# Autodesk Inventor assembly: V1Flywheel
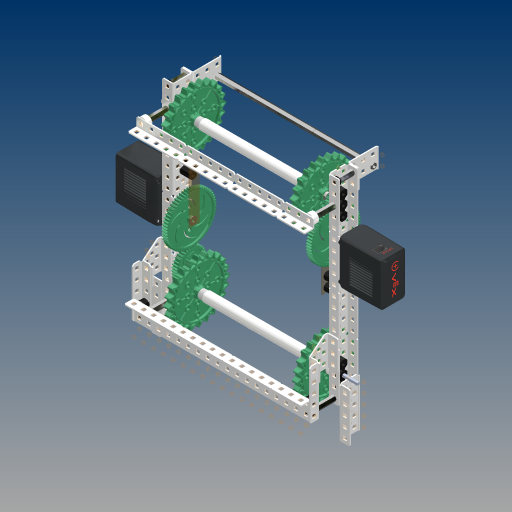
[picture p0: Inventor's stored thumbnail of the model, 512x512]
Saved by Autodesk Inventor 2023 (Build 270158000, 158)
## iProperties
Created: 2023-07-16
Part Number: V1Flywheel
Document SubType Name: Assembly
Designer: eddie
Author: eddie
## Documents named in this file (35)
- C:\Users\eddie\Documents\81208X-Over-Under-CAD\V1\V1Flywheel.iam
- C:\Users\eddie\Documents\81208X-Over-Under-CAD\VEX-CAD-Inventor-1.4.0\Structure\C Channel\Aluminum 1x2x1\Alu C 1x2x1x20.ipt
- C:\Users\eddie\Documents\81208X-Over-Under-CAD\VEX-CAD-Inventor-1.4.0\Motion\Shaft LS\Bearing Flat.ipt
- C:\Users\eddie\Documents\81208X-Over-Under-CAD\VEX-CAD-Inventor-1.4.0\Electronics\V5 Motor.ipt
- C:\Users\eddie\Documents\81208X-Over-Under-CAD\VEX-CAD-Inventor-1.4.0\Structure\Standoff\Standoff 1.00.ipt
- C:\Users\eddie\Documents\81208X-Over-Under-CAD\VEX-CAD-Inventor-1.4.0\Structure\Standoff.ipt
- C:\Users\eddie\Documents\81208X-Over-Under-CAD\VEX-CAD-Inventor-1.4.0\Motion\Spacers\Spacer Nylon .500 OD\NSpacer White .500 OD x .250.ipt
- C:\Users\eddie\Documents\81208X-Over-Under-CAD\VEX-CAD-Inventor-1.4.0\Motion\Spacers\Spacer Nylon .500 OD.ipt
- C:\Users\eddie\Documents\81208X-Over-Under-CAD\VEX-CAD-Inventor-1.4.0\Structure\Angle\Aluminum\1x1\Alu Angle 1x1x18.ipt
- C:\Users\eddie\Documents\81208X-Over-Under-CAD\VEX-CAD-Inventor-1.4.0\Motion\Shaft LS\Shaft LS\Shaft LS 9.0.ipt
- C:\Users\eddie\Documents\81208X-Over-Under-CAD\VEX-CAD-Inventor-1.4.0\Motion\Shaft LS\Shaft LS.ipt
- C:\Users\eddie\Documents\81208X-Over-Under-CAD\Custom-parts\Shaft Collar.ipt
- C:\Users\eddie\Documents\81208X-Over-Under-CAD\VEX-CAD-Inventor-1.4.0\Motion\Sprockets\9P Sprocket\9P 24T Sprocket, Square.iam
- C:\Users\eddie\Documents\81208X-Over-Under-CAD\VEX-CAD-Inventor-1.4.0\Motion\Sprockets\9P Sprocket.iam
- C:\Users\eddie\Documents\81208X-Over-Under-CAD\VEX-CAD-Inventor-1.4.0\Motion\Spacers\Spacer Nylon .500 OD\NSpacer White .500 OD x .375.ipt
- C:\Users\eddie\Documents\81208X-Over-Under-CAD\VEX-CAD-Inventor-1.4.0\Motion\Spacers\Washer Steel\SWasher .375 OD x .031250.ipt
- C:\Users\eddie\Documents\81208X-Over-Under-CAD\VEX-CAD-Inventor-1.4.0\Motion\Spacers\Washer Steel.ipt
- C:\Users\eddie\Documents\81208X-Over-Under-CAD\VEX-CAD-Inventor-1.4.0\Motion\Gears\LS 12T Gear.ipt
- C:\Users\eddie\Documents\81208X-Over-Under-CAD\VEX-CAD-Inventor-1.4.0\Motion\Gears\LS 60T Gear.ipt
- C:\Users\eddie\Documents\81208X-Over-Under-CAD\VEX-CAD-Inventor-1.4.0\Motion\Spacers\Spacer Nylon .375 OD\NSpacer .375 OD x .125.ipt
- C:\Users\eddie\Documents\81208X-Over-Under-CAD\VEX-CAD-Inventor-1.4.0\Motion\Spacers\Spacer Nylon .375 OD.ipt
- C:\Users\eddie\Documents\81208X-Over-Under-CAD\VEX-CAD-Inventor-1.4.0\Motion\Gears\LS 36T Gear.ipt
- C:\Users\eddie\Documents\81208X-Over-Under-CAD\VEX-CAD-Inventor-1.4.0\Motion\Gears\LS 12T Gear Steel.ipt
- C:\Users\eddie\Documents\81208X-Over-Under-CAD\VEX-CAD-Inventor-1.4.0\Structure\Angle\Aluminum\1x1\Alu Angle 1x1x5.ipt
- C:\Users\eddie\Documents\81208X-Over-Under-CAD\VEX-CAD-Inventor-1.4.0\Motion\Spacers\Spacer Nylon .375 OD\NSpacer .375 OD x .250.ipt
- C:\Users\eddie\Documents\81208X-Over-Under-CAD\Custom-parts\3x3x18 channel minus halfcut.ipt
- C:\Users\eddie\Documents\81208X-Over-Under-CAD\Custom-parts\3x2 channel triangular slice.ipt
- C:\Users\eddie\Documents\81208X-Over-Under-CAD\Custom-parts\2x3 channel without 1 side.ipt
- C:\Users\eddie\Documents\81208X-Over-Under-CAD\VEX-CAD-Inventor-1.4.0\Structure\Standoff\Standoff .75.ipt
- C:\Users\eddie\Documents\81208X-Over-Under-CAD\VEX-CAD-Inventor-1.4.0\Structure\Standoff\Standoff 5.00.ipt
- C:\Users\eddie\Documents\81208X-Over-Under-CAD\VEX-CAD-Inventor-1.4.0\Structure\Standoff\Standoff 3.00.ipt
- C:\Users\eddie\Documents\81208X-Over-Under-CAD\Custom-parts\2x5 channel without 1 side.ipt
- C:\Users\eddie\Documents\81208X-Over-Under-CAD\VEX-CAD-Inventor-1.4.0\Structure\Hardware\Nut Nylock.ipt
- C:\Users\eddie\Documents\81208X-Over-Under-CAD\Custom-parts\6holepolycarb.ipt
- C:\Users\eddie\Documents\81208X-Over-Under-CAD\VEX-CAD-Inventor-1.4.0\Motion\Spacers\Spacer Nylon .375 OD\NSpacer .375 OD x .375.ipt
## Components (119 placed, 28 different names)
1. Alu C 1x2x1x20:1 — Insert:1, Insert:2, Insert:3, Insert:36, Insert:71, Insert:72, Insert:91, Insert:92, Insert:96, Insert:119, Insert:120
2. Bearing Flat:1 — Insert:1, Insert:10
3. V5 Motor:1 — Insert:2
4. Standoff 1.00:1 — Insert:3, Insert:4
5. NSpacer White .500 OD x .250:1 — Insert:4, Insert:5
6. Alu Angle 1x1x18:1 — Insert:5, Insert:6
7. NSpacer White .500 OD x .250:2 — Insert:6, Insert:7
8. Standoff 1.00:2 — Insert:7, Insert:8
9. Alu C 1x2x1x20:2 — Insert:8, Insert:9, Insert:11, Insert:39, Insert:40, Insert:41, Insert:42, Insert:44, Insert:47, Insert:80, Insert:90, Insert:93, Insert:98, Insert:114, Mate:1
10. Bearing Flat:2 — Insert:9
11. Shaft LS 9.0:1 — Insert:10
12. NSpacer White .500 OD x .250:3 — Insert:11, Insert:12
13. Shaft Collar:1 — Insert:13, Insert:14
14. 9P 24T Sprocket, Square:1 [sub-assembly] — Insert:12, Insert:13
15. NSpacer White .500 OD x .250:4 — Insert:14, Insert:15
16. NSpacer White .500 OD x .375:5 — Insert:15, Insert:16
17. NSpacer White .500 OD x .375:6 — Insert:18, Insert:19
18. NSpacer White .500 OD x .375:7 — Insert:21, Insert:22
19. NSpacer White .500 OD x .375:8 — Insert:19, Insert:20
20. NSpacer White .500 OD x .375:9 — Insert:17, Insert:18
21. NSpacer White .500 OD x .375:10 — Insert:16, Insert:17
22. NSpacer White .500 OD x .375:11 — Insert:24, Insert:25
23. NSpacer White .500 OD x .375:12 — Insert:22, Insert:23
24. NSpacer White .500 OD x .375:13 — Insert:25, Insert:26
25. NSpacer White .500 OD x .375:14 — Insert:23, Insert:24
26. NSpacer White .500 OD x .375:15 — Insert:26, Insert:27
27. NSpacer White .500 OD x .375:16 — Insert:27, Insert:28
28. NSpacer White .500 OD x .375:17 — Insert:20, Insert:21
29. NSpacer White .500 OD x .375:18 — Insert:28, Insert:29
30. Shaft Collar:2 — Insert:29, Insert:30
31. 9P 24T Sprocket, Square:2 [sub-assembly] — Insert:30, Insert:31
32. SWasher .375 OD x .031250:1 — Insert:31, Insert:32
33. SWasher .375 OD x .031250:2 — Insert:32, Insert:33
34. SWasher .375 OD x .031250:3 — Insert:34, Insert:35
35. SWasher .375 OD x .031250:4 — Insert:33, Insert:34
36. LS 12T Gear:1 — Insert:35
37. SWasher .375 OD x .031250:5 — Insert:36, Insert:37
38. LS 60T Gear:1 — Insert:37, Insert:123
39. Bearing Flat:3 — Insert:39, Insert:46, Insert:109
40. Bearing Flat:4 — Insert:40
41. V5 Motor:2 — Insert:41
42. NSpacer .375 OD x .125:1 — Insert:42, Insert:43
43. LS 60T Gear:2 — Insert:43, Insert:112
44. LS 36T Gear:1 — Insert:45
45. NSpacer .375 OD x .125:2 — Insert:44, Insert:45
46. Shaft LS 9.0:2 — Insert:46
47. LS 12T Gear Steel:1 — Insert:47, Insert:48
48. SWasher .375 OD x .031250:6 — Insert:48, Insert:49
49. SWasher .375 OD x .031250:7 — Insert:49, Insert:50
50. 9P 24T Sprocket, Square:3 [sub-assembly] — Insert:50, Insert:51
51. Shaft Collar:3 — Insert:51, Insert:52
52. NSpacer White .500 OD x .375:19 — Insert:52, Insert:53
53. NSpacer White .500 OD x .375:20 — Insert:53, Insert:54
54. NSpacer White .500 OD x .375:21 — Insert:54, Insert:55
55. NSpacer White .500 OD x .375:22 — Insert:55, Insert:56
56. NSpacer White .500 OD x .375:23 — Insert:57, Insert:58
57. NSpacer White .500 OD x .375:24 — Insert:56, Insert:57
58. NSpacer White .500 OD x .250:25 — Insert:58, Insert:59
59. NSpacer White .500 OD x .375:26 — Insert:59, Insert:60
60. NSpacer White .500 OD x .375:27 — Insert:60, Insert:61
61. NSpacer White .500 OD x .375:28 — Insert:61, Insert:62
62. NSpacer White .500 OD x .375:29 — Insert:62, Insert:63
63. NSpacer White .500 OD x .375:30 — Insert:63, Insert:64
64. NSpacer White .500 OD x .375:31 — Insert:64, Insert:65
65. NSpacer White .500 OD x .375:32 — Insert:66, Insert:67
66. NSpacer White .500 OD x .375:33 — Insert:65, Insert:66
67. Shaft Collar:4 — Insert:67, Insert:68
68. 9P 24T Sprocket, Square:4 [sub-assembly] — Insert:68, Insert:69
69. NSpacer White .500 OD x .250:34 — Insert:69
70. Bearing Flat:5 — Insert:71, Insert:106
71. Standoff 1.00:3 — Insert:72, Insert:73
72. Alu Angle 1x1x5:1 — Insert:73, Insert:74, Insert:75
73. NSpacer .375 OD x .250:3 — Insert:76, Insert:78
74. NSpacer .375 OD x .250:4 — Insert:77, Insert:79
75. SWasher .375 OD x .031250:8 — Insert:79
76. SWasher .375 OD x .031250:9 — Insert:75, Insert:77
77. SWasher .375 OD x .031250:10 — Insert:74, Insert:76
78. SWasher .375 OD x .031250:11 — Insert:78
79. Standoff 1.00:4 — Insert:80, Insert:82
80. Alu Angle 1x1x5:2 — Insert:82, Insert:83, Insert:84
81. SWasher .375 OD x .031250:12 — Insert:84, Insert:86
82. SWasher .375 OD x .031250:13 — Insert:83, Insert:85
83. SWasher .375 OD x .031250:14 — Insert:87
84. SWasher .375 OD x .031250:15 — Insert:88, Insert:89
85. NSpacer .375 OD x .250:5 — Insert:86, Insert:88
86. NSpacer .375 OD x .250:6 — Insert:85, Insert:87
87. 3x3x18 channel minus halfcut:1 — Insert:89
88. 3x2 channel triangular slice:1 — Insert:90
89. 3x2 channel triangular slice:2 — Insert:91
90. 2x3 channel without 1 side:1 — Insert:92
91. 2x3 channel without 1 side:2 — Insert:93, Insert:100
92. NSpacer .375 OD x .125:8 — Insert:96, Insert:97
93. Standoff .75:6 — Insert:97
94. NSpacer .375 OD x .125:9 — Insert:98, Insert:99
95. Standoff .75:7 — Insert:99
96. Standoff 5.00:8 — Insert:100, Insert:101
97. Standoff 3.00:9 — Insert:101
98. 2x5 channel without 1 side:1 — Insert:108
99. Nut Nylock:1 — Insert:106, Insert:107
100. SWasher .375 OD x .031250:18 — Insert:107, Insert:108
101. Nut Nylock:2 — Insert:109, Insert:110
102. SWasher .375 OD x .031250:19 — Insert:110, Insert:111
103. 2x5 channel without 1 side:2 — Insert:111
104. SWasher .375 OD x .031250:20 — Insert:112, Insert:113
105. 6holepolycarb:1 — Insert:113
106. SWasher .375 OD x .031250:22 — Insert:114, Insert:116
107. SWasher .375 OD x .031250:24 — Mate:1, Insert:115
108. NSpacer .375 OD x .375:10 — Insert:115, Insert:118
109. NSpacer .375 OD x .375:11 — Insert:116, Insert:117
110. NSpacer .375 OD x .125:12 — Insert:118
111. NSpacer .375 OD x .125:13 — Insert:117
112. SWasher .375 OD x .031250:25 — Insert:120, Insert:122
113. SWasher .375 OD x .031250:26 — Insert:119, Insert:121
114. NSpacer .375 OD x .375:14 — Insert:121, Insert:125
115. NSpacer .375 OD x .375:15 — Insert:122, Insert:126
116. 6holepolycarb:2 — Insert:124
117. NSpacer .375 OD x .125:16 — Insert:123, Insert:124
118. NSpacer .375 OD x .125:17 — Insert:125
119. NSpacer .375 OD x .125:18 — Insert:126
## Relationships (118: Insert 117, Mate 1)
- Insert:1: Alu C 1x2x1x20:1 ↔ Bearing Flat:1
- Insert:2: Alu C 1x2x1x20:1 ↔ V5 Motor:1
- Insert:3: Alu C 1x2x1x20:1 ↔ Standoff 1.00:1
- Insert:4: Standoff 1.00:1 ↔ NSpacer White .500 OD x .250:1
- Insert:5: NSpacer White .500 OD x .250:1 ↔ Alu Angle 1x1x18:1
- Insert:6: Alu Angle 1x1x18:1 ↔ NSpacer White .500 OD x .250:2
- Insert:7: NSpacer White .500 OD x .250:2 ↔ Standoff 1.00:2
- Insert:8: Standoff 1.00:2 ↔ Alu C 1x2x1x20:2
- Insert:9: Alu C 1x2x1x20:2 ↔ Bearing Flat:2
- Insert:10: Bearing Flat:1 ↔ Shaft LS 9.0:1
- Insert:11: Alu C 1x2x1x20:2 ↔ NSpacer White .500 OD x .250:3
- Insert:12: NSpacer White .500 OD x .250:3 ↔ 9P 24T Sprocket, Square:1
- Insert:13: Shaft Collar:1 ↔ 9P 24T Sprocket, Square:1
- Insert:14: Shaft Collar:1 ↔ NSpacer White .500 OD x .250:4
- Insert:15: NSpacer White .500 OD x .250:4 ↔ NSpacer White .500 OD x .375:5
- Insert:16: NSpacer White .500 OD x .375:5 ↔ NSpacer White .500 OD x .375:10
- Insert:17: NSpacer White .500 OD x .375:9 ↔ NSpacer White .500 OD x .375:10
- Insert:18: NSpacer White .500 OD x .375:6 ↔ NSpacer White .500 OD x .375:9
- Insert:19: NSpacer White .500 OD x .375:6 ↔ NSpacer White .500 OD x .375:8
- Insert:20: NSpacer White .500 OD x .375:8 ↔ NSpacer White .500 OD x .375:17
- Insert:21: NSpacer White .500 OD x .375:7 ↔ NSpacer White .500 OD x .375:17
- Insert:22: NSpacer White .500 OD x .375:7 ↔ NSpacer White .500 OD x .375:12
- Insert:23: NSpacer White .500 OD x .375:12 ↔ NSpacer White .500 OD x .375:14
- Insert:24: NSpacer White .500 OD x .375:11 ↔ NSpacer White .500 OD x .375:14
- Insert:25: NSpacer White .500 OD x .375:11 ↔ NSpacer White .500 OD x .375:13
- Insert:26: NSpacer White .500 OD x .375:13 ↔ NSpacer White .500 OD x .375:15
- Insert:27: NSpacer White .500 OD x .375:15 ↔ NSpacer White .500 OD x .375:16
- Insert:28: NSpacer White .500 OD x .375:16 ↔ NSpacer White .500 OD x .375:18
- Insert:29: NSpacer White .500 OD x .375:18 ↔ Shaft Collar:2
- Insert:30: Shaft Collar:2 ↔ 9P 24T Sprocket, Square:2
- Insert:31: 9P 24T Sprocket, Square:2 ↔ SWasher .375 OD x .031250:1
- Insert:32: SWasher .375 OD x .031250:1 ↔ SWasher .375 OD x .031250:2
- Insert:33: SWasher .375 OD x .031250:2 ↔ SWasher .375 OD x .031250:4
- Insert:34: SWasher .375 OD x .031250:3 ↔ SWasher .375 OD x .031250:4
- Insert:35: SWasher .375 OD x .031250:3 ↔ LS 12T Gear:1
- Insert:36: Alu C 1x2x1x20:1 ↔ SWasher .375 OD x .031250:5
- Insert:37: SWasher .375 OD x .031250:5 ↔ LS 60T Gear:1
- Insert:39: Alu C 1x2x1x20:2 ↔ Bearing Flat:3
- Insert:40: Alu C 1x2x1x20:2 ↔ Bearing Flat:4
- Insert:41: Alu C 1x2x1x20:2 ↔ V5 Motor:2
- Insert:42: Alu C 1x2x1x20:2 ↔ NSpacer .375 OD x .125:1
- Insert:43: NSpacer .375 OD x .125:1 ↔ LS 60T Gear:2
- Insert:44: Alu C 1x2x1x20:2 ↔ NSpacer .375 OD x .125:2
- Insert:45: LS 36T Gear:1 ↔ NSpacer .375 OD x .125:2
- Insert:46: Bearing Flat:3 ↔ Shaft LS 9.0:2
- Insert:47: Alu C 1x2x1x20:2 ↔ LS 12T Gear Steel:1
- Insert:48: LS 12T Gear Steel:1 ↔ SWasher .375 OD x .031250:6
- Insert:49: SWasher .375 OD x .031250:6 ↔ SWasher .375 OD x .031250:7
- Insert:50: SWasher .375 OD x .031250:7 ↔ 9P 24T Sprocket, Square:3
- Insert:51: 9P 24T Sprocket, Square:3 ↔ Shaft Collar:3
- Insert:52: Shaft Collar:3 ↔ NSpacer White .500 OD x .375:19
- Insert:53: NSpacer White .500 OD x .375:19 ↔ NSpacer White .500 OD x .375:20
- Insert:54: NSpacer White .500 OD x .375:20 ↔ NSpacer White .500 OD x .375:21
- Insert:55: NSpacer White .500 OD x .375:21 ↔ NSpacer White .500 OD x .375:22
- Insert:56: NSpacer White .500 OD x .375:22 ↔ NSpacer White .500 OD x .375:24
- Insert:57: NSpacer White .500 OD x .375:23 ↔ NSpacer White .500 OD x .375:24
- Insert:58: NSpacer White .500 OD x .375:23 ↔ NSpacer White .500 OD x .250:25
- Insert:59: NSpacer White .500 OD x .250:25 ↔ NSpacer White .500 OD x .375:26
- Insert:60: NSpacer White .500 OD x .375:26 ↔ NSpacer White .500 OD x .375:27
- Insert:61: NSpacer White .500 OD x .375:27 ↔ NSpacer White .500 OD x .375:28
- Insert:62: NSpacer White .500 OD x .375:28 ↔ NSpacer White .500 OD x .375:29
- Insert:63: NSpacer White .500 OD x .375:29 ↔ NSpacer White .500 OD x .375:30
- Insert:64: NSpacer White .500 OD x .375:30 ↔ NSpacer White .500 OD x .375:31
- Insert:65: NSpacer White .500 OD x .375:31 ↔ NSpacer White .500 OD x .375:33
- Insert:66: NSpacer White .500 OD x .375:32 ↔ NSpacer White .500 OD x .375:33
- Insert:67: NSpacer White .500 OD x .375:32 ↔ Shaft Collar:4
- Insert:68: Shaft Collar:4 ↔ 9P 24T Sprocket, Square:4
- Insert:69: 9P 24T Sprocket, Square:4 ↔ NSpacer White .500 OD x .250:34
- Insert:71: Alu C 1x2x1x20:1 ↔ Bearing Flat:5
- Insert:72: Alu C 1x2x1x20:1 ↔ Standoff 1.00:3
- Insert:73: Standoff 1.00:3 ↔ Alu Angle 1x1x5:1
- Insert:74: Alu Angle 1x1x5:1 ↔ SWasher .375 OD x .031250:10
- Insert:75: Alu Angle 1x1x5:1 ↔ SWasher .375 OD x .031250:9
- Insert:76: NSpacer .375 OD x .250:3 ↔ SWasher .375 OD x .031250:10
- Insert:77: NSpacer .375 OD x .250:4 ↔ SWasher .375 OD x .031250:9
- Insert:78: NSpacer .375 OD x .250:3 ↔ SWasher .375 OD x .031250:11
- Insert:79: NSpacer .375 OD x .250:4 ↔ SWasher .375 OD x .031250:8
- Insert:80: Alu C 1x2x1x20:2 ↔ Standoff 1.00:4
- Insert:82: Standoff 1.00:4 ↔ Alu Angle 1x1x5:2
- Insert:83: Alu Angle 1x1x5:2 ↔ SWasher .375 OD x .031250:13
- Insert:84: Alu Angle 1x1x5:2 ↔ SWasher .375 OD x .031250:12
- Insert:85: SWasher .375 OD x .031250:13 ↔ NSpacer .375 OD x .250:6
- Insert:86: SWasher .375 OD x .031250:12 ↔ NSpacer .375 OD x .250:5
- Insert:87: SWasher .375 OD x .031250:14 ↔ NSpacer .375 OD x .250:6
- Insert:88: SWasher .375 OD x .031250:15 ↔ NSpacer .375 OD x .250:5
- Insert:89: SWasher .375 OD x .031250:15 ↔ 3x3x18 channel minus halfcut:1
- Insert:90: Alu C 1x2x1x20:2 ↔ 3x2 channel triangular slice:1
- Insert:91: Alu C 1x2x1x20:1 ↔ 3x2 channel triangular slice:2
- Insert:92: Alu C 1x2x1x20:1 ↔ 2x3 channel without 1 side:1
- Insert:93: Alu C 1x2x1x20:2 ↔ 2x3 channel without 1 side:2
- Insert:96: Alu C 1x2x1x20:1 ↔ NSpacer .375 OD x .125:8
- Insert:97: NSpacer .375 OD x .125:8 ↔ Standoff .75:6
- Insert:98: Alu C 1x2x1x20:2 ↔ NSpacer .375 OD x .125:9
- Insert:99: NSpacer .375 OD x .125:9 ↔ Standoff .75:7
- Insert:100: 2x3 channel without 1 side:2 ↔ Standoff 5.00:8
- Insert:101: Standoff 5.00:8 ↔ Standoff 3.00:9
- Insert:106: Bearing Flat:5 ↔ Nut Nylock:1
- Insert:107: Nut Nylock:1 ↔ SWasher .375 OD x .031250:18
- Insert:108: 2x5 channel without 1 side:1 ↔ SWasher .375 OD x .031250:18
- Insert:109: Bearing Flat:3 ↔ Nut Nylock:2
- Insert:110: Nut Nylock:2 ↔ SWasher .375 OD x .031250:19
- Insert:111: SWasher .375 OD x .031250:19 ↔ 2x5 channel without 1 side:2
- Insert:112: LS 60T Gear:2 ↔ SWasher .375 OD x .031250:20
- Insert:113: SWasher .375 OD x .031250:20 ↔ 6holepolycarb:1
- Insert:114: Alu C 1x2x1x20:2 ↔ SWasher .375 OD x .031250:22
- Mate:1: Alu C 1x2x1x20:2 ↔ SWasher .375 OD x .031250:24
- Insert:115: SWasher .375 OD x .031250:24 ↔ NSpacer .375 OD x .375:10
- Insert:116: SWasher .375 OD x .031250:22 ↔ NSpacer .375 OD x .375:11
- Insert:117: NSpacer .375 OD x .375:11 ↔ NSpacer .375 OD x .125:13
- Insert:118: NSpacer .375 OD x .375:10 ↔ NSpacer .375 OD x .125:12
- Insert:119: Alu C 1x2x1x20:1 ↔ SWasher .375 OD x .031250:26
- Insert:120: Alu C 1x2x1x20:1 ↔ SWasher .375 OD x .031250:25
- Insert:121: SWasher .375 OD x .031250:26 ↔ NSpacer .375 OD x .375:14
- Insert:122: SWasher .375 OD x .031250:25 ↔ NSpacer .375 OD x .375:15
- Insert:123: LS 60T Gear:1 ↔ NSpacer .375 OD x .125:16
- Insert:124: 6holepolycarb:2 ↔ NSpacer .375 OD x .125:16
- Insert:125: NSpacer .375 OD x .375:14 ↔ NSpacer .375 OD x .125:17
- Insert:126: NSpacer .375 OD x .375:15 ↔ NSpacer .375 OD x .125:18
